# Autodesk Inventor assembly: 20220613_機体完成
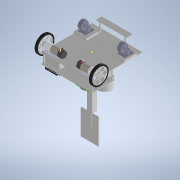
[picture p0: Inventor's stored thumbnail of the model, 180x180]
Saved by Autodesk Inventor 2020 (Build 240168000, 168)
## iProperties
Created: 2022-06-13
Part Number: 20220613_機体完成
Document SubType Name: Assembly
Designer: Naggy
Author: Naggy
## Documents named in this file (19)
- C:\Users\Naggy\Documents\Inventor\robot_design2020\20220613_機体完成.iam
- C:\Users\Naggy\Documents\Inventor\robot_design2020\202205026_知能ロボ1階部分.ipt
- C:\Users\Naggy\Documents\Inventor\robot_design2020\20220519モータを取り付けるやつ.ipt
- C:\Users\Naggy\Documents\Inventor\robot_design2020\20220519知能ロボットモータとエンコーダ.ipt
- C:\Users\Naggy\Documents\Inventor\robot_design2020\70アルミホイール内径4.ipt
- C:\Users\Naggy\Documents\Inventor\robot_design2020\20220509_知能ロボットキャスタ.ipt
- C:\Users\Naggy\Documents\Inventor\robot_design2020\RD003_キャスタ420G-R32 (3).ipt
- C:\Users\Naggy\Documents\Inventor\robot_design2020\20220527知能ロボットスペーサ.ipt
- C:\Users\Naggy\Documents\Inventor\robot_design2020\20220526_知能ロボ2階部分.ipt
- C:\Users\Naggy\Documents\Inventor\robot_design2020\20220530_カメラ支え完成.ipt
- C:\Users\Naggy\Documents\Inventor\robot_design2020\20220523_センサモジュール.ipt
- C:\Users\Naggy\Documents\Inventor\robot_design2020\20220523_arduinoMEGA.ipt
- C:\Users\Naggy\Documents\Inventor\robot_design2020\20220523_Raspberry_Pi.ipt
- C:\Users\Naggy\Documents\Inventor\robot_design2020\202200606_知能ロボットanker.ipt
- C:\Users\Naggy\Documents\Inventor\robot_design2020\tamiya_sporttuned.ipt
- C:\Users\Naggy\Documents\Inventor\robot_design2020\20220613_筒.ipt
- C:\Users\Naggy\Documents\Inventor\robot_design2020\20220610_サーボ仮.ipt
- C:\Users\Naggy\Documents\Inventor\robot_design2020\20220613_サーボ固定.ipt
- C:\Users\Naggy\Documents\Inventor\robot_design2020\20220613_カメラ固定.ipt
## Components (28 placed, 18 different names)
1. 202205026_知能ロボ1階部分:1 — メイト:1, メイト:2, メイト:3, メイト:8, メイト:9, メイト:12, メイト:13, メイト:14, メイト:15, メイト:16, メイト:17, メイト:19, メイト:26, 挿入:1
2. 20220519モータを取り付けるやつ:1 — メイト:2, メイト:5
3. 20220519モータを取り付けるやつ:2 — メイト:3, メイト:4
4. 20220519知能ロボットモータとエンコーダ:1 — メイト:4, メイト:6
5. 20220519知能ロボットモータとエンコーダ:2 — メイト:5, メイト:7
6. 70アルミホイール内径4:1 — メイト:7
7. 70アルミホイール内径4:2 — メイト:6
8. 20220509_知能ロボットキャスタ:1 — メイト:8, メイト:11
9. 20220509_知能ロボットキャスタ:2 — メイト:9, メイト:10
10. RD003_キャスタ420G-R32 (3):1 — メイト:11
11. RD003_キャスタ420G-R32 (3):2 — メイト:10
12. 20220527知能ロボットスペーサ:1 — メイト:12, メイト:22
13. 20220527知能ロボットスペーサ:2 — メイト:13
14. 20220527知能ロボットスペーサ:3 — メイト:14
15. 20220527知能ロボットスペーサ:4 — メイト:15
16. 20220527知能ロボットスペーサ:5 — メイト:17
17. 20220527知能ロボットスペーサ:6 — メイト:16, メイト:21
18. 20220530_カメラ支え完成:1 — メイト:19, メイト:28
19. 20220523_センサモジュール:1 — メイト:21
20. 20220523_arduinoMEGA:3 — メイト:23
21. 20220523_Raspberry_Pi:6 — メイト:24
22. 20220526_知能ロボ2階部分:1 — メイト:22, メイト:23, メイト:24
23. 202200606_知能ロボットanker:1 — メイト:26
24. 20220610_サーボ仮:1 — 挿入:1, 挿入:2
25. 20220613_筒:1 — 挿入:3, メイト:27
26. tamiya_sporttuned:1 — メイト:27
27. 20220613_サーボ固定:1 — 挿入:2, 挿入:3
28. 20220613_カメラ固定:2 — メイト:28
## Relationships (28: Mate 25, Insert 3)
- メイト:1 [Mate]: 202205026_知能ロボ1階部分:1
- メイト:2 [Mate]: 202205026_知能ロボ1階部分:1 ↔ 20220519モータを取り付けるやつ:1
- メイト:3 [Mate]: 202205026_知能ロボ1階部分:1 ↔ 20220519モータを取り付けるやつ:2
- メイト:4 [Mate]: 20220519モータを取り付けるやつ:2 ↔ 20220519知能ロボットモータとエンコーダ:1
- メイト:5 [Mate]: 20220519モータを取り付けるやつ:1 ↔ 20220519知能ロボットモータとエンコーダ:2
- メイト:6 [Mate]: 20220519知能ロボットモータとエンコーダ:1 ↔ 70アルミホイール内径4:2
- メイト:7 [Mate]: 20220519知能ロボットモータとエンコーダ:2 ↔ 70アルミホイール内径4:1
- メイト:8 [Mate]: 202205026_知能ロボ1階部分:1 ↔ 20220509_知能ロボットキャスタ:1
- メイト:9 [Mate]: 202205026_知能ロボ1階部分:1 ↔ 20220509_知能ロボットキャスタ:2
- メイト:10 [Mate]: 20220509_知能ロボットキャスタ:2 ↔ RD003_キャスタ420G-R32 (3):2
- メイト:11 [Mate]: 20220509_知能ロボットキャスタ:1 ↔ RD003_キャスタ420G-R32 (3):1
- メイト:12 [Mate]: 202205026_知能ロボ1階部分:1 ↔ 20220527知能ロボットスペーサ:1
- メイト:13 [Mate]: 202205026_知能ロボ1階部分:1 ↔ 20220527知能ロボットスペーサ:2
- メイト:14 [Mate]: 202205026_知能ロボ1階部分:1 ↔ 20220527知能ロボットスペーサ:3
- メイト:15 [Mate]: 202205026_知能ロボ1階部分:1 ↔ 20220527知能ロボットスペーサ:4
- メイト:16 [Mate]: 202205026_知能ロボ1階部分:1 ↔ 20220527知能ロボットスペーサ:6
- メイト:17 [Mate]: 202205026_知能ロボ1階部分:1 ↔ 20220527知能ロボットスペーサ:5
- メイト:19 [Mate]: 202205026_知能ロボ1階部分:1 ↔ 20220530_カメラ支え完成:1
- メイト:21 [Mate]: 20220527知能ロボットスペーサ:6 ↔ 20220523_センサモジュール:1
- メイト:22 [Mate]: 20220527知能ロボットスペーサ:1 ↔ 20220526_知能ロボ2階部分:1
- メイト:23 [Mate]: 20220523_arduinoMEGA:3 ↔ 20220526_知能ロボ2階部分:1
- メイト:24 [Mate]: 20220523_Raspberry_Pi:6 ↔ 20220526_知能ロボ2階部分:1
- メイト:26 [Mate]: 202205026_知能ロボ1階部分:1 ↔ 202200606_知能ロボットanker:1
- 挿入:1 [Insert]: 202205026_知能ロボ1階部分:1 ↔ 20220610_サーボ仮:1
- 挿入:2 [Insert]: 20220610_サーボ仮:1 ↔ 20220613_サーボ固定:1
- 挿入:3 [Insert]: 20220613_筒:1 ↔ 20220613_サーボ固定:1
- メイト:27 [Mate]: 20220613_筒:1 ↔ tamiya_sporttuned:1
- メイト:28 [Mate]: 20220530_カメラ支え完成:1 ↔ 20220613_カメラ固定:2
